# Autodesk Inventor assembly: One Motor Plate
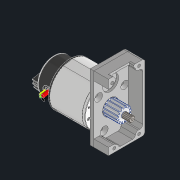
[picture p0: Inventor's stored thumbnail of the model, 180x180]
Saved by Autodesk Inventor 2022 (Build 260153000, 153)
## iProperties
Created: 2022-09-09
Part Number: One Motor Plate
Document SubType Name: Assembly
Designer: robpl
Author: robpl
## Documents named in this file (4)
- C:\Users\robpl\OneDrive\Documents\Inventor\2022 FRC Season\Best Coast Drive\Left One Motor Plate.iam
- C:\Users\robpl\OneDrive\Documents\Inventor\2022 FRC Season\Best Coast Drive\Left One Motor Plate.ipt
- C:\Users\robpl\OneDrive\Documents\Inventor\2022 FRC Season\Best Coast Drive\Falcon 500, Powered by Talon FX (217-6515).ipt
- C:\Users\robpl\OneDrive\Documents\Inventor\2022 FRC Season\Best Coast Drive\Left One Motor Gearbox Cover.ipt
## Components (3 placed, 3 different names)
1. Left One Motor Plate:1 — Mate:1, Mate:2, Mate:5, Mate:6, Flush:1, Flush:2
2. Falcon 500, Powered by Talon FX (217-6515):1 — Mate:1, Mate:2, Mate:5
3. Left One Motor Gearbox Cover:1 — Mate:6, Flush:1, Flush:2
## Relationships (6: Mate 4, Flush 2)
- Mate:1: Left One Motor Plate:1 ↔ Falcon 500, Powered by Talon FX (217-6515):1
- Mate:2: Left One Motor Plate:1 ↔ Falcon 500, Powered by Talon FX (217-6515):1
- Mate:5: Left One Motor Plate:1 ↔ Falcon 500, Powered by Talon FX (217-6515):1
- Mate:6: Left One Motor Plate:1 ↔ Left One Motor Gearbox Cover:1
- Flush:1: Left One Motor Plate:1 ↔ Left One Motor Gearbox Cover:1
- Flush:2: Left One Motor Plate:1 ↔ Left One Motor Gearbox Cover:1
